# Autodesk Inventor assembly: 頭_1_2
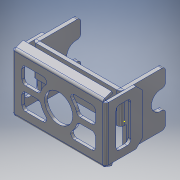
[picture p0: Inventor's stored thumbnail of the model, 180x180]
Saved by Autodesk Inventor 2018 (Build 220112000, 112)
## iProperties
Created: 2016-05-10
Part Number: 頭_1_2
Document SubType Name: Assembly
Designer: hiroaki
Mass: 17.9103 g
Surface Area: 119.086 cm^2
Volume: 7.5268 cm^3
Density: 2.37954 g/cm^3
Author: hiroaki
## Documents named in this file (3)
- C:\Users\taka\Desktop\OPR\OpenPlatform_ver1_0\上半身\頭\頭_1_2.iam
- C:\Users\taka\Desktop\OPR\OpenPlatform_ver1_0\上半身\頭\頭_メインフレーム_1_2.ipt
- C:\Users\taka\Desktop\OPR\OpenPlatform_ver1_0\上半身\頭\頭_メインフレーム_1_4.ipt
## Components (2 placed, 2 different names)
1. 頭_メインフレーム_1_2:1 — メイト:4, メイト:5, メイト:6
2. 頭_メインフレーム_1_4:1 — メイト:4, メイト:5, メイト:6
## Relationships (3: Mate 3)
- メイト:4 [Mate]: 頭_メインフレーム_1_2:1 ↔ 頭_メインフレーム_1_4:1
- メイト:5 [Mate]: 頭_メインフレーム_1_2:1 ↔ 頭_メインフレーム_1_4:1
- メイト:6 [Mate]: 頭_メインフレーム_1_2:1 ↔ 頭_メインフレーム_1_4:1
